# Autodesk Inventor assembly: SentiBot
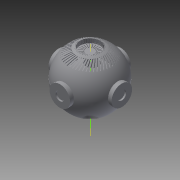
[picture p0: Inventor's stored thumbnail of the model, 180x180]
Saved by Autodesk Inventor 2015 (Build 190159000, 159)
## iProperties
Created: 2015-07-02
Part Number: SentiBot
Document SubType Name: Assembly
Designer: Sudhar
Author: Sudhar
## Documents named in this file (4)
- C:\Users\Sudhar\Computer Documents\Desktop\IRP\SentiBot.iam
- C:\Users\Sudhar\Computer Documents\Desktop\IRP\SentiBot botton.ipt
- C:\Users\Sudhar\Computer Documents\Desktop\IRP\SentiBot top.ipt
- C:\Users\Sudhar\Computer Documents\Desktop\IRP\connectors.ipt
## Components (6 placed, 3 different names)
1. SentiBot botton:1
2. SentiBot top:1
3. connectors:1
4. connectors:2
5. connectors:3
6. connectors:4
## Component patterns: (4 elements, first: connectors:1)
